# Autodesk Inventor assembly: HitecServoAssembly
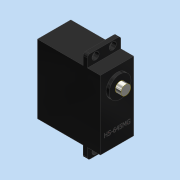
[picture p0: Inventor's stored thumbnail of the model, 180x180]
Saved by Autodesk Inventor 2017 (Build 210142000, 142)
## iProperties
Created: 2016-10-23
Part Number: HitecServoAssembly
Document SubType Name: Assembly
Designer: techn
Mass: 56.699 g
Surface Area: 68.7297 cm^2
Volume: 30.4214 cm^3
Author: techn
## Documents named in this file (3)
- G:\Projects\Submarine\Submarine-project\CAD\common\HitecServo\HitecServoAssembly.iam
- G:\Projects\Submarine\Submarine-project\CAD\common\HitecServo\HitecServoBody.ipt
- G:\Projects\Submarine\Submarine-project\CAD\common\HitecServo\HitecServoNub.ipt
## Components (2 placed, 2 different names)
1. HitecServoBody:1 — Mate:1, Mate:2
2. HitecServoNub:1 — Mate:1, Mate:2
## Relationships (2: Mate 2)
- Mate:1: HitecServoBody:1 ↔ HitecServoNub:1
- Mate:2: HitecServoBody:1 ↔ HitecServoNub:1
